# Autodesk Inventor assembly: ASY Beshkino_bio_tank
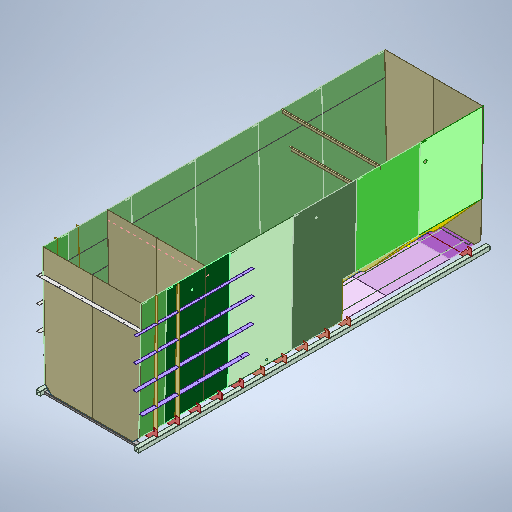
[picture p0: Inventor's stored thumbnail of the model, 512x512]
Saved by Autodesk Inventor 2025 (Build 290162010, 162A)
## iProperties
Created: 2024-07-21
Part Number: ASY Beshkino_bio_tank
Document SubType Name: Assembly
Designer: admin
Mass: 5.81287e+06 g
Surface Area: 2.77755e+06 cm^2
Volume: 3.12018e+06 cm^3
Density: 1.86299 g/cm^3
Author: admin
## Documents named in this file (35)
- C:\Users\pokla\Documents\Inventor\BSH_Beshkino_bio_tank\ASY Beshkino_bio_tank.iam
- C:\Users\pokla\Documents\Inventor\BSH_Beshkino_bio_tank\BSH 000 dim Beshkino_bio_tank.ipt
- C:\Users\pokla\Documents\Inventor\BSH_Beshkino_bio_tank\BSH 010 floor 1.ipt
- C:\Users\pokla\Documents\Inventor\BSH_Beshkino_bio_tank\BSH 021 rib 1.ipt
- C:\Users\pokla\Documents\Inventor\BSH_Beshkino_bio_tank\BSH 022 rib 2.ipt
- C:\Users\pokla\Documents\Inventor\BSH_Beshkino_bio_tank\BSH 061 tube 1.ipt
- C:\Users\pokla\Documents\Inventor\BSH_Beshkino_bio_tank\BSH 031 nose 1.ipt
- C:\Users\pokla\Documents\Inventor\BSH_Beshkino_bio_tank\BSH 032 board 2.ipt
- C:\Users\pokla\Documents\Inventor\BSH_Beshkino_bio_tank\BSH 033 board 3.ipt
- C:\Users\pokla\Documents\Inventor\BSH_Beshkino_bio_tank\BSH 041 stringer 1.ipt
- C:\Users\pokla\Documents\Inventor\BSH_Beshkino_bio_tank\BSH 039 back 9.ipt
- C:\Users\pokla\Documents\Inventor\BSH_Beshkino_bio_tank\BSH 041 stringer floor.ipt
- C:\Users\pokla\Documents\Inventor\BSH_Beshkino_bio_tank\BSH 062 tube 2.ipt
- C:\Users\pokla\Documents\Inventor\BSH_Beshkino_bio_tank\BSH 042 stringer 2.ipt
- C:\Users\pokla\Documents\Inventor\BSH_Beshkino_bio_tank\BSH 043 stringer 3.ipt
- C:\Users\pokla\Documents\Inventor\BSH_Beshkino_bio_tank\BSH 044 stringer 4.ipt
- C:\Users\pokla\Documents\Inventor\BSH_Beshkino_bio_tank\BSH 042 stringer floor.ipt
- C:\Users\pokla\Documents\Inventor\BSH_Beshkino_bio_tank\BSH 045 stringer 1.ipt
- C:\Users\pokla\Documents\Inventor\BSH_Beshkino_bio_tank\BSH 045 stringer 5.ipt
- C:\Users\pokla\Documents\Inventor\BSH_Beshkino_bio_tank\BSH 033 board cone 3.ipt
- C:\Users\pokla\Documents\Inventor\BSH_Beshkino_bio_tank\BSH 034 board cone 4.ipt
- C:\Users\pokla\Documents\Inventor\BSH_Beshkino_bio_tank\BSH 035 divider 1.ipt
- C:\Users\pokla\Documents\Inventor\BSH_Beshkino_bio_tank\BSH 036 divider 2.ipt
- C:\Users\pokla\Documents\Inventor\BSH_Beshkino_bio_tank\BSH 012 floor 2.ipt
- C:\Users\pokla\Documents\Inventor\BSH_Beshkino_bio_tank\BSH 037 cone 3.ipt
- C:\Users\pokla\Documents\Inventor\BSH_Beshkino_bio_tank\BSH 013 floor 3.ipt
- C:\Users\pokla\Documents\Inventor\BSH_Beshkino_bio_tank\BSH 015 board cone 5.ipt
- C:\Users\pokla\Documents\Inventor\BSH_Beshkino_bio_tank\BSH 038 divider.ipt
- C:\Users\pokla\Documents\Inventor\BSH_Beshkino_bio_tank\BSH 046 stringer 6.ipt
- C:\Users\pokla\Documents\Inventor\BSH_Beshkino_bio_tank\BSH 035 board cone 5.ipt
- C:\Users\pokla\Documents\Inventor\BSH_Beshkino_bio_tank\BSH 035 board .ipt
- C:\Users\pokla\Documents\Inventor\BSH_Beshkino_bio_tank\BSH 051 back 1.ipt
- C:\Users\pokla\Documents\Inventor\BSH_Beshkino_bio_tank\BSH 052 board 2.ipt
- C:\Users\pokla\Documents\Inventor\BSH_Beshkino_bio_tank\BSH 053 board 3.ipt
- C:\Users\pokla\Documents\Inventor\BSH_Beshkino_bio_tank\BSH 054 board cone 4.ipt
## Components (86 placed, 40 different names)
1. BSH 000 dim Beshkino_bio_tank.ipt:1
2. BSH 022 rib 2.ipt:1 — Rigid:27, Rigid:28, Rigid:29, Rigid:30, Rigid:74
3. BSH 061 tube 1.ipt:1 — Mate:1, Rigid:1, Mate:3, Flush:12, Mate:66, Mate:67
4. BSH 061 tube 1.ipt:2 — Mate:2, Rigid:1, Mate:4, Flush:3, Flush:4, Flush:16, Mate:65, Flush:20
5. BSH 062 tube 2.ipt:1 — Mate:19, Flush:12, Flush:16, Mate:65
6. BSH 062 tube 2.ipt:2 — Mate:68, Flush:20
7. BSH 010 floor 1.ipt:2 — Rigid:5, Rigid:83, Mate:77, Flush:18, Flush:19
8. BSH 010 floor 1.ipt:3 — Rigid:5, Rigid:82
9. BSH 010 floor 1.ipt:1 — Mate:5, Mate:6, Mate:7, Flush:4, Mate:10, Flush:5, Flush:11, Flush:17, Mate:70, Rigid:82, Mate:74
10. BSH 031 nose 1.ipt:1 — Mate:10, Flush:5, Mate:11, Rigid:11, Mate:58, Mate:73
11. BSH 033 board 3.ipt:1 — Flush:11, Mate:73, Mate:74, Rigid:104
12. BSH 031 nose 1.ipt:2 — Rigid:11, Rigid:53, Mate:69
13. BSH 021 rib 1.ipt:1 — Mate:4, Flush:3, Mate:5, Mate:6, Rigid:9, Rigid:20, Rigid:22, Rigid:24, Rigid:26, Mate:19, Rigid:74, Rigid:76
14. BSH 041 stringer floor.ipt:2 — Rigid:22
15. BSH 041 stringer floor.ipt:3 — Rigid:24
16. BSH 041 stringer floor.ipt:4 — Rigid:26
17. BSH 041 stringer floor.ipt:5 — Rigid:95
18. BSH 041 stringer floor.ipt:6
19. BSH 041 stringer floor:10 — Rigid:96
20. BSH 041 stringer floor:11
21. BSH 041 stringer floor:12 — Rigid:97
22. BSH 041 stringer floor:14 — Rigid:98, Rigid:99, Rigid:100, Rigid:101, Rigid:102
23. BSH 041 stringer floor:13
24. BSH 041 stringer floor:15
25. BSH 041 stringer floor.ipt:1 — Rigid:20, Rigid:91, Rigid:92, Rigid:93
26. BSH 042 stringer floor:1 — Rigid:87
27. BSH 042 stringer floor:2 — Rigid:86
28. BSH 042 stringer floor:3 — Rigid:85
29. BSH 042 stringer floor:4 — Rigid:84
30. BSH 045 stringer 1:1
31. BSH 045 stringer 5:1 — Mate:22, Mate:23
32. BSH 031 nose 1:3 — Mate:22
33. BSH 031 nose 1:4 — Rigid:53
34. BSH 033 board cone 3:1 — Mate:26, Rigid:57, Mate:30, Mate:80, Mate:83
35. BSH 031 nose 1:7 — Mate:26, Mate:30, Mate:84, Flush:21
36. BSH 031 nose 1:8 — Flush:8, Mate:40
37. BSH 033 board cone 3:2 — Rigid:57, Angle:1, Mate:49, Mate:50, Mate:64, Mate:71
38. BSH 043 stringer 3.ipt:1 — Rigid:29
39. BSH 042 stringer 2.ipt:1 — Rigid:28
40. BSH 041 stringer 1.ipt:1 — Rigid:27
41. BSH 041 stringer 1.ipt:2
42. BSH 042 stringer 2.ipt:2
43. BSH 043 stringer 3.ipt:2
44. BSH 044 stringer 4.ipt:2 — Mate:59, Flush:13, Flush:15, Rigid:71
45. BSH 034 board cone 4:2 — Mate:84, Rigid:108, Mate:88, Mate:89, Mate:90, Mate:91
46. BSH 035 divider 1:1 — Mate:44
47. BSH 036 divider 2:1
48. BSH 012 floor 2:1 — Rigid:66, Mate:42, Angle:1, Mate:49, Rigid:83, Mate:72, Mate:87
49. BSH 037 cone 3:1 — Mate:42, Mate:50, Mate:90
50. BSH 033 board 3:2 — Flush:17, Mate:69, Mate:70, Rigid:81
51. BSH 012 floor 2:2 — Rigid:66, Rigid:67, Mate:63, Mate:78
52. BSH 013 floor 3:1 — Rigid:67, Mate:40, Mate:81
53. BSH 039 back 9:2 — Rigid:90, Rigid:103
54. BSH 015 board cone 5:1 — Mate:71, Mate:72, Mate:85, Mate:86
55. BSH 038 divider:1 — Mate:77, Flush:18, Flush:19
56. BSH 046 stringer 6:1 — Mate:58, Mate:59, Flush:13, Flush:15
57. BSH 037 cone 3:2 — Mate:63, Mate:64, Mate:91
58. BSH 044 stringer 4:3 — Rigid:71, Rigid:72
59. BSH 044 stringer 4:4 — Rigid:72
60. BSH 022 rib 2:34 — Rigid:76
61. BSH 020 rib 1:4 — Mate:66, Mate:67, Mate:68, Rigid:84, Rigid:85, Rigid:86, Rigid:87
62. BSH 022 rib 2:35 — Rigid:77
63. BSH 021 rib 1.ipt:2 — Rigid:9, Rigid:75, Rigid:77
64. BSH 037 cone 3:3 — Mate:78, Mate:80, Mate:88
65. BSH 037 cone 3:4 — Mate:81, Mate:83, Mate:89
66. BSH 035 board cone 5:1 — Rigid:107
67. BSH 035 board :1 — Rigid:90, Mate:85, Rigid:106
68. BSH 020 rib 1:5 — Rigid:91
69. BSH 020 rib 1:6 — Rigid:92
70. BSH 020 rib 1:7 — Rigid:93, Rigid:94
71. BSH 020 rib 1:8 — Rigid:94, Rigid:95, Rigid:96, Rigid:97, Rigid:98
72. BSH 020 rib 1:9 — Rigid:99
73. BSH 020 rib 1:10 — Rigid:100
74. BSH 020 rib 1:11 — Rigid:101
75. BSH 020 rib 1:12 — Rigid:102
76. BSH 051 back 1:1 — Rigid:103, Flush:21
77. BSH 052 board 2:1 — Rigid:104, Rigid:105
78. BSH 044 stringer 4.ipt:1 — Rigid:30
79. BSH 022 rib 2:33 — Rigid:75
80. BSH 053 board 3:1 — Rigid:105, Rigid:106
81. BSH 054 board cone 4:1 — Rigid:107, Rigid:108, Mate:86, Mate:87
82. BSH 032 board 2:4 — Rigid:81
83. BSH 032 board 2:5
84. BSH 032 board 2:6
85. BSH 032 board 2:7
86. BSH 032 board 2:8
## Component patterns: (5 elements, first: BSH 032 board 2:4)
## Relationships (111: WeldJoint 50, Mate 46, Flush 14, Angle 1)
- Mate:1: BSH 061 tube 1.ipt:1
- Mate:2: BSH 061 tube 1.ipt:2
- Rigid:1 [WeldJoint] (-2400 mm): BSH 061 tube 1.ipt:1 ↔ BSH 061 tube 1.ipt:2
- Mate:3: BSH 061 tube 1.ipt:1
- Mate:4: BSH 061 tube 1.ipt:2 ↔ BSH 021 rib 1.ipt:1
- Flush:3: BSH 061 tube 1.ipt:2 ↔ BSH 021 rib 1.ipt:1
- Mate:5: BSH 010 floor 1.ipt:1 ↔ BSH 021 rib 1.ipt:1
- Mate:6: BSH 010 floor 1.ipt:1 ↔ BSH 021 rib 1.ipt:1
- Rigid:5 [WeldJoint]: BSH 010 floor 1.ipt:2 ↔ BSH 010 floor 1.ipt:3
- Mate:7: BSH 010 floor 1.ipt:1
- Flush:4 (100 mm): BSH 061 tube 1.ipt:2 ↔ BSH 010 floor 1.ipt:1
- Rigid:9 [WeldJoint] (-500 mm): BSH 021 rib 1.ipt:1 ↔ BSH 021 rib 1.ipt:2
- Mate:10: BSH 010 floor 1.ipt:1 ↔ BSH 031 nose 1.ipt:1
- Flush:5 (10 mm): BSH 010 floor 1.ipt:1 ↔ BSH 031 nose 1.ipt:1
- Mate:11: BSH 031 nose 1.ipt:1
- Rigid:11 [WeldJoint]: BSH 031 nose 1.ipt:1 ↔ BSH 031 nose 1.ipt:2
- Rigid:20 [WeldJoint] (2 mm): BSH 021 rib 1.ipt:1 ↔ BSH 041 stringer floor.ipt:1
- Rigid:22 [WeldJoint] (2 mm): BSH 021 rib 1.ipt:1 ↔ BSH 041 stringer floor.ipt:2
- Rigid:24 [WeldJoint] (2 mm): BSH 021 rib 1.ipt:1 ↔ BSH 041 stringer floor.ipt:3
- Rigid:26 [WeldJoint] (2 mm): BSH 021 rib 1.ipt:1 ↔ BSH 041 stringer floor.ipt:4
- Rigid:27 [WeldJoint] (2 mm): BSH 022 rib 2.ipt:1 ↔ BSH 041 stringer 1.ipt:1
- Rigid:28 [WeldJoint] (2 mm): BSH 022 rib 2.ipt:1 ↔ BSH 042 stringer 2.ipt:1
- Rigid:29 [WeldJoint] (2 mm): BSH 022 rib 2.ipt:1 ↔ BSH 043 stringer 3.ipt:1
- Rigid:30 [WeldJoint] (2 mm): BSH 022 rib 2.ipt:1 ↔ BSH 044 stringer 4.ipt:1
- Mate:19 (248.5 mm): BSH 062 tube 2.ipt:1 ↔ BSH 021 rib 1.ipt:1
- Mate:22: BSH 045 stringer 5:1 ↔ BSH 031 nose 1:3
- Mate:23: BSH 045 stringer 5:1
- [WeldJoint]: BSH 031 nose 1:3 ↔ BSH 031 nose 1:4
- Rigid:53 [WeldJoint] (1500 mm): BSH 031 nose 1.ipt:2 ↔ BSH 031 nose 1:4
- [WeldJoint]: BSH 031 nose 1:7 ↔ BSH 031 nose 1:8
- Flush:8: BSH 031 nose 1:8
- Mate:26: BSH 033 board cone 3:1 ↔ BSH 031 nose 1:7
- Rigid:57 [WeldJoint]: BSH 033 board cone 3:1 ↔ BSH 033 board cone 3:2
- Mate:30: BSH 033 board cone 3:1 ↔ BSH 031 nose 1:7
- Flush:11: BSH 010 floor 1.ipt:1 ↔ BSH 033 board 3.ipt:1
- Rigid:66 [WeldJoint]: BSH 012 floor 2:1 ↔ BSH 012 floor 2:2
- Rigid:67 [WeldJoint]: BSH 012 floor 2:2 ↔ BSH 013 floor 3:1
- Mate:40: BSH 031 nose 1:8 ↔ BSH 013 floor 3:1
- Mate:42: BSH 012 floor 2:1 ↔ BSH 037 cone 3:1
- Mate:44: BSH 035 divider 1:1
- Angle:1 (132 deg): BSH 033 board cone 3:2 ↔ BSH 012 floor 2:1
- Mate:49: BSH 033 board cone 3:2 ↔ BSH 012 floor 2:1
- Mate:50: BSH 033 board cone 3:2 ↔ BSH 037 cone 3:1
- Mate:58: BSH 031 nose 1.ipt:1 ↔ BSH 046 stringer 6:1
- Flush:12: BSH 061 tube 1.ipt:1 ↔ BSH 062 tube 2.ipt:1
- Mate:59: BSH 044 stringer 4.ipt:2 ↔ BSH 046 stringer 6:1
- Flush:13 (10 mm): BSH 044 stringer 4.ipt:2 ↔ BSH 046 stringer 6:1
- Mate:63: BSH 012 floor 2:2 ↔ BSH 037 cone 3:2
- Mate:64: BSH 033 board cone 3:2 ↔ BSH 037 cone 3:2
- Flush:15 (5 mm): BSH 044 stringer 4.ipt:2 ↔ BSH 046 stringer 6:1
- Rigid:71 [WeldJoint] (-10 mm): BSH 044 stringer 4.ipt:2 ↔ BSH 044 stringer 4:3
- Rigid:72 [WeldJoint] (-10 mm): BSH 044 stringer 4:3 ↔ BSH 044 stringer 4:4
- Rigid:74 [WeldJoint] (-10 mm): BSH 022 rib 2.ipt:1 ↔ BSH 021 rib 1.ipt:1
- Flush:16 (90 mm): BSH 061 tube 1.ipt:2 ↔ BSH 062 tube 2.ipt:1
- Mate:65: BSH 061 tube 1.ipt:2 ↔ BSH 062 tube 2.ipt:1
- Rigid:75 [WeldJoint] (-10 mm): BSH 021 rib 1.ipt:2 ↔ BSH 022 rib 2:33
- Rigid:76 [WeldJoint] (-10 mm): BSH 021 rib 1.ipt:1 ↔ BSH 022 rib 2:34
- Rigid:77 [WeldJoint] (-10 mm): BSH 022 rib 2:35 ↔ BSH 021 rib 1.ipt:2
- Mate:66: BSH 061 tube 1.ipt:1 ↔ BSH 020 rib 1:4
- Mate:67: BSH 061 tube 1.ipt:1 ↔ BSH 020 rib 1:4
- Mate:68 (248.5 mm): BSH 062 tube 2.ipt:2 ↔ BSH 020 rib 1:4
- Flush:17: BSH 010 floor 1.ipt:1 ↔ BSH 033 board 3:2
- Mate:69: BSH 031 nose 1.ipt:2 ↔ BSH 033 board 3:2
- Mate:70: BSH 010 floor 1.ipt:1 ↔ BSH 033 board 3:2
- Rigid:81 [WeldJoint]: BSH 033 board 3:2 ↔ BSH 032 board 2:4
- Rigid:82 [WeldJoint]: BSH 010 floor 1.ipt:3 ↔ BSH 010 floor 1.ipt:1
- Rigid:83 [WeldJoint]: BSH 010 floor 1.ipt:2 ↔ BSH 012 floor 2:1
- Rigid:84 [WeldJoint] (2 mm): BSH 042 stringer floor:4 ↔ BSH 020 rib 1:4
- Rigid:85 [WeldJoint] (2 mm): BSH 042 stringer floor:3 ↔ BSH 020 rib 1:4
- Rigid:86 [WeldJoint] (2 mm): BSH 042 stringer floor:2 ↔ BSH 020 rib 1:4
- Rigid:87 [WeldJoint] (2 mm): BSH 042 stringer floor:1 ↔ BSH 020 rib 1:4
- Mate:71: BSH 033 board cone 3:2 ↔ BSH 015 board cone 5:1
- Mate:72: BSH 012 floor 2:1 ↔ BSH 015 board cone 5:1
- Mate:73: BSH 031 nose 1.ipt:1 ↔ BSH 033 board 3.ipt:1
- Mate:74: BSH 010 floor 1.ipt:1 ↔ BSH 033 board 3.ipt:1
- Mate:77: BSH 010 floor 1.ipt:2 ↔ BSH 038 divider:1
- Flush:18: BSH 010 floor 1.ipt:2 ↔ BSH 038 divider:1
- Flush:19: BSH 010 floor 1.ipt:2 ↔ BSH 038 divider:1
- Mate:78: BSH 012 floor 2:2 ↔ BSH 037 cone 3:3
- Mate:80: BSH 033 board cone 3:1 ↔ BSH 037 cone 3:3
- Mate:81: BSH 013 floor 3:1 ↔ BSH 037 cone 3:4
- Mate:83: BSH 033 board cone 3:1 ↔ BSH 037 cone 3:4
- Mate:84: BSH 031 nose 1:7 ↔ BSH 034 board cone 4:2
- Rigid:90 [WeldJoint]: BSH 039 back 9:2 ↔ BSH 035 board :1
- Mate:85: BSH 015 board cone 5:1 ↔ BSH 035 board :1
- Rigid:91 [WeldJoint] (2 mm): BSH 041 stringer floor.ipt:1 ↔ BSH 020 rib 1:5
- Rigid:92 [WeldJoint] (2 mm): BSH 041 stringer floor.ipt:1 ↔ BSH 020 rib 1:6
- Rigid:93 [WeldJoint] (2 mm): BSH 041 stringer floor.ipt:1 ↔ BSH 020 rib 1:7
- Rigid:94 [WeldJoint] (500 mm): BSH 020 rib 1:7 ↔ BSH 020 rib 1:8
- Rigid:95 [WeldJoint] (2 mm): BSH 041 stringer floor.ipt:5 ↔ BSH 020 rib 1:8
- Rigid:96 [WeldJoint] (2 mm): BSH 041 stringer floor:10 ↔ BSH 020 rib 1:8
- Rigid:97 [WeldJoint] (2 mm): BSH 041 stringer floor:12 ↔ BSH 020 rib 1:8
- Rigid:98 [WeldJoint] (2 mm): BSH 041 stringer floor:14 ↔ BSH 020 rib 1:8
- Rigid:99 [WeldJoint] (2 mm): BSH 041 stringer floor:14 ↔ BSH 020 rib 1:9
- Rigid:100 [WeldJoint] (2 mm): BSH 041 stringer floor:14 ↔ BSH 020 rib 1:10
- Rigid:101 [WeldJoint] (2 mm): BSH 041 stringer floor:14 ↔ BSH 020 rib 1:11
- Rigid:102 [WeldJoint] (2 mm): BSH 041 stringer floor:14 ↔ BSH 020 rib 1:12
- Flush:20: BSH 061 tube 1.ipt:2 ↔ BSH 062 tube 2.ipt:2
- Rigid:103 [WeldJoint]: BSH 039 back 9:2 ↔ BSH 051 back 1:1
- Rigid:104 [WeldJoint]: BSH 033 board 3.ipt:1 ↔ BSH 052 board 2:1
- Rigid:105 [WeldJoint]: BSH 052 board 2:1 ↔ BSH 053 board 3:1
- Rigid:106 [WeldJoint]: BSH 035 board :1 ↔ BSH 053 board 3:1
- Flush:21 (10 mm): BSH 031 nose 1:7 ↔ BSH 051 back 1:1
- Rigid:107 [WeldJoint]: BSH 035 board cone 5:1 ↔ BSH 054 board cone 4:1
- Rigid:108 [WeldJoint]: BSH 034 board cone 4:2 ↔ BSH 054 board cone 4:1
- Mate:86: BSH 015 board cone 5:1 ↔ BSH 054 board cone 4:1
- Mate:87: BSH 012 floor 2:1 ↔ BSH 054 board cone 4:1
- Mate:88: BSH 034 board cone 4:2 ↔ BSH 037 cone 3:3
- Mate:89: BSH 034 board cone 4:2 ↔ BSH 037 cone 3:4
- Mate:90: BSH 034 board cone 4:2 ↔ BSH 037 cone 3:1
- Mate:91: BSH 034 board cone 4:2 ↔ BSH 037 cone 3:2
## Named parameters: d118_d31 = 0 mm, d124_d31 = 0 mm
